# Autodesk Inventor assembly: Molde_completo
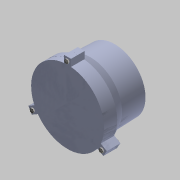
[picture p0: Inventor's stored thumbnail of the model, 180x180]
Saved by Autodesk Inventor 2019 (Build 230136000, 136)
## iProperties
Created: 2019-05-29
Part Number: Molde_completo
Document SubType Name: Assembly
Designer: Emily Rojas
Author: Emily Rojas
## Documents named in this file (5)
- C:\Users\gusta\Documents\UPB\Diseño\Actividad 5\Pieza_1\Molde_completo.iam
- C:\Users\gusta\Documents\UPB\Diseño\Actividad 5\Pieza_1\Molde_Exterior.ipt
- C:\Users\gusta\Documents\UPB\Diseño\Actividad 5\Pieza_1\Molde_Interior.ipt
- C:\Users\gusta\Documents\UPB\Diseño\Actividad 5\Pieza_1\AS 1110 - M5 x 35.ipt
- C:\Users\gusta\Documents\UPB\Diseño\Actividad 5\Pieza_1\AS 1112 - M5(2).ipt
## Components (8 placed, 4 different names)
1. Molde_Exterior:1 — Flush:1, Flush:2, Mate:1, Mate:2, Mate:3, Mate:4, Mate:5, Mate:6, Mate:7
2. Molde_Interior:1 — Flush:1, Flush:2, Mate:1, Mate:8, Mate:9, Mate:10
3. AS 1110 - Metric M5 x 35:1 — Mate:2, Mate:7, Mate:11
4. AS 1110 - Metric M5 x 35:2 — Mate:3, Mate:6, Mate:13
5. AS 1110 - Metric M5 x 35:3 — Mate:4, Mate:5, Mate:12
6. AS 1112 (4) - Metric M5:1 — Mate:8, Mate:11
7. AS 1112 (4) - Metric M5:2 — Mate:9, Mate:12
8. AS 1112 (4) - Metric M5:3 — Mate:10, Mate:13
## Relationships (15: Mate 13, Flush 2)
- Flush:1: Molde_Exterior:1 ↔ Molde_Interior:1
- Flush:2: Molde_Exterior:1 ↔ Molde_Interior:1
- Mate:1: Molde_Exterior:1 ↔ Molde_Interior:1
- Mate:2: Molde_Exterior:1 ↔ AS 1110 - Metric M5 x 35:1
- Mate:3: Molde_Exterior:1 ↔ AS 1110 - Metric M5 x 35:2
- Mate:4: Molde_Exterior:1 ↔ AS 1110 - Metric M5 x 35:3
- Mate:5: Molde_Exterior:1 ↔ AS 1110 - Metric M5 x 35:3
- Mate:6: Molde_Exterior:1 ↔ AS 1110 - Metric M5 x 35:2
- Mate:7: Molde_Exterior:1 ↔ AS 1110 - Metric M5 x 35:1
- Mate:8: Molde_Interior:1 ↔ AS 1112 (4) - Metric M5:1
- Mate:9: Molde_Interior:1 ↔ AS 1112 (4) - Metric M5:2
- Mate:10: Molde_Interior:1 ↔ AS 1112 (4) - Metric M5:3
- Mate:11: AS 1110 - Metric M5 x 35:1 ↔ AS 1112 (4) - Metric M5:1
- Mate:12: AS 1110 - Metric M5 x 35:3 ↔ AS 1112 (4) - Metric M5:2
- Mate:13: AS 1110 - Metric M5 x 35:2 ↔ AS 1112 (4) - Metric M5:3
